# Autodesk Inventor assembly: servoMoldAssembly
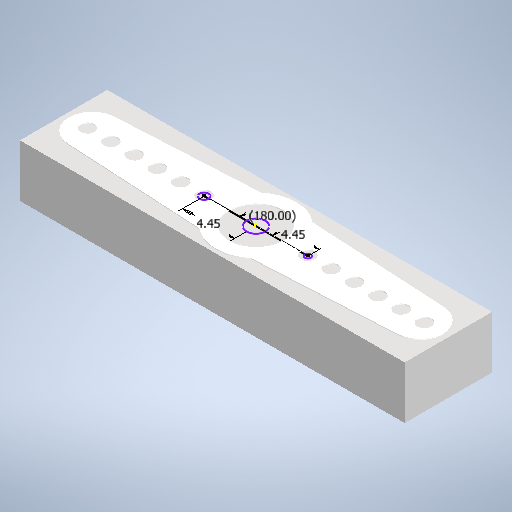
[picture p0: Inventor's stored thumbnail of the model, 512x512]
Saved by Autodesk Inventor 2025.1 (Build 291241020, 241B)
## iProperties
Created: 2025-03-17
Part Number: servoMoldAssembly
Document SubType Name: Assembly
Designer: omiye
Author: omiye
## Documents named in this file (3)
- C:\Projects\Arduino\MazeRobot\models\sg90\servoMoldAssembly.iam
- C:\Projects\Arduino\MazeRobot\models\sg90\block.ipt
- C:\Projects\Arduino\MazeRobot\models\sg90\sg90horn.ipt
## Components (2 placed, 2 different names)
1. block:1 — Mate:1, Mate:2, Mate:3
2. sg90horn:1 — Mate:1, Mate:2, Mate:3
## Relationships (3: Mate 3)
- Mate:1: block:1 ↔ sg90horn:1
- Mate:2: block:1 ↔ sg90horn:1
- Mate:3: block:1 ↔ sg90horn:1
